# Autodesk Inventor assembly: boardstack
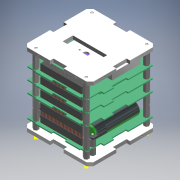
[picture p0: Inventor's stored thumbnail of the model, 180x180]
Saved by Autodesk Inventor 2022.3 (Build 263350000, 350)
## iProperties
Created: 2021-10-07
Part Number: boardstack
Document SubType Name: Assembly
Designer: Bowen O'Steen
Mass: 647.8 g
Surface Area: 2149.86 cm^2
Volume: 273.038 cm^3
Density: 2.37256 g/cm^3
Author: Bowen O'Steen
## Documents named in this file (11)
- C:\Users\gwhen\OneDrive\Documents\Vault\Engineering Data\MemeSat\Assembly\boardstack.iam
- C:\Users\gwhen\OneDrive\Desktop\Vault\Designs\MEMESat\MemeSat\Engineering Data\MemeSat\Subsystems\LFR\fullLFRboard.iam
- C:\Users\gwhen\OneDrive\Desktop\Vault\Designs\MEMESat\MemeSat\Engineering Data\MemeSat\Subsystems\OBC\OBC.iam
- C:\Users\gwhen\OneDrive\Desktop\Vault\Designs\MEMESat\MemeSat\Engineering Data\MemeSat\Subsystems\BoBa\BoBa.iam
- C:\Users\gwhen\OneDrive\Desktop\Vault\Designs\MEMESat\MemeSat\Engineering Data\MemeSat\Internal Components\pc104standoff.ipt
- C:\Users\gwhen\OneDrive\Desktop\Vault\Designs\MEMESat\MemeSat\Engineering Data\MemeSat\Subsystems\fullPCIconnector.iam
- C:\Users\gwhen\OneDrive\Desktop\Vault\Designs\MEMESat\MemeSat\Engineering Data\MemeSat\Subsystems\blankPC104plus.iam
- C:\Users\gwhen\OneDrive\Desktop\Vault\Designs\MEMESat\MemeSat\Engineering Data\MemeSat\Internal Components\stackframesupport.ipt
- C:\Users\gwhen\OneDrive\Desktop\Vault\Designs\MEMESat\MemeSat\Engineering Data\MemeSat\Internal Components\stackframesupportbottom.ipt
- C:\Users\gwhen\OneDrive\Desktop\Vault\Designs\MEMESat\MemeSat\Engineering Data\MemeSat\Internal Components\pc104standoffTEMP.ipt
- C:\Users\gwhen\OneDrive\Desktop\Vault\Designs\MEMESat\MemeSat\Engineering Data\MemeSat\Internal Components\pcBOBAstandoff.ipt
## Components (43 placed, 9 different names)
1. fullLFRboard:1 [sub-assembly] — Flush:1, Flush:2, Flush:3, Mate:1, Mate:2, Mate:3, Mate:4, Mate:5, Mate:6, Mate:7, Mate:8, Mate:46, Mate:47, Mate:61
2. OBC:1 [sub-assembly] — Mate:9, Mate:10, Mate:11, Mate:12, Mate:13, Mate:14, Mate:15, Mate:16, Mate:17, Mate:18, Mate:19, Angle:5, Angle:6, Angle:7, Angle:8
3. blankPC104plus:1 [sub-assembly] — Mate:20, Mate:21, Mate:22, Mate:23, Mate:24, Mate:25, Mate:26, Mate:31, Mate:32, Mate:33, Mate:34, Mate:43, Mate:44, Mate:45, Angle:9, Angle:10, Angle:11, Angle:12, Flush:6, Angle:13, Angle:20
4. pc104standoff:1 — Mate:1, Mate:8, Angle:5, Flush:8
5. pc104standoff:2 — Mate:2, Mate:7, Mate:9, Mate:10, Angle:6, Flush:9
6. pc104standoff:3 — Mate:3, Mate:5, Mate:11, Angle:8, Flush:10, Mate:60
7. pc104standoff:4 — Mate:4, Mate:6, Angle:7, Flush:7
8. pc104standoff:5 — Mate:12, Mate:17, Mate:20, Mate:22, Angle:10
9. pc104standoff:6 — Mate:13, Mate:16, Mate:21, Angle:9
10. pc104standoff:7 — Mate:14, Mate:19, Angle:11
11. pc104standoff:8 — Mate:15, Mate:18, Angle:12
12. pc104standoff:9 — Mate:26, Mate:30, Mate:32, Mate:37, Angle:13, Angle:14
13. pc104standoff:10 — Mate:24, Mate:28, Mate:34, Mate:36, Angle:23
14. pc104standoff:11 — Mate:23, Mate:29, Mate:31, Mate:35, Angle:20
15. pc104standoff:12 — Mate:25, Mate:27, Mate:33, Mate:38, Angle:24
16. pc104standoff:13 — Mate:27, Mate:38, Flush:14, Angle:24
17. pc104standoff:14 — Mate:28, Mate:36, Flush:11, Angle:23
18. pc104standoff:15 — Mate:29, Mate:35, Flush:12, Angle:21
19. pc104standoff:16 — Mate:30, Mate:37, Flush:13, Mate:50, Angle:14
20. fullPCIconnector:1 [sub-assembly] — Mate:43, Mate:44, Mate:45, Flush:5
21. stackframesupport:2 — Insert:1, Insert:2, Insert:3
22. stackframesupportbottom:1 — Insert:7, Insert:8, Insert:9, Insert:10, Insert:11, Mate:54, Mate:55
23. pc104standoff:21
24. pc104standoff:22
25. pc104standoff:23
26. pc104standoff:24
27. BoBa:1 [sub-assembly] — Flush:5, Flush:6, Insert:4, Insert:5, Insert:6, Mate:49, Mate:50, Mate:51, Angle:15, Angle:16, Mate:53, Angle:17, Mate:57, Mate:59, Angle:18, Angle:19, Angle:21, Angle:22
28. pcLFRstandoff:1 — Insert:1, Flush:7
29. pcLFRstandoff:2 — Insert:2, Flush:8, Mate:47
30. pcLFRstandoff:3 — Insert:3, Flush:9, Mate:46
31. pcLFRstandoff:4 — Flush:10, Mate:60, Mate:61
32. pcLFRstandoff:5 — Insert:4, Flush:11, Insert:7, Flush:15
33. pcLFRstandoff:6 — Insert:6, Flush:13
34. pcLFRstandoff:7 — Flush:14, Flush:16, Mate:54, Mate:55
35. pcLFRstandoff:8 — Insert:5, Flush:12, Angle:22
36. pcLFRstandoff:9 — Insert:8, Flush:15, Mate:56
37. pcLFRstandoff:10 — Insert:9, Flush:16, Mate:52
38. pcLFRstandoff:11 — Insert:11, Mate:58, Angle:19
39. pcLFRstandoff:12 — Insert:10, Mate:48, Mate:51, Angle:16
40. pcLFRstandoff:13 — Mate:48, Mate:49, Angle:15
41. pcLFRstandoff:14 — Mate:52, Mate:53, Angle:17
42. pcLFRstandoff:15 — Mate:56, Mate:57
43. pcLFRstandoff:16 — Mate:58, Mate:59, Angle:18
## Relationships (103: Mate 57, Angle 20, Flush 15, Insert 11)
- Flush:1: fullLFRboard:1
- Flush:2: fullLFRboard:1
- Flush:3: fullLFRboard:1
- Mate:1: fullLFRboard:1 ↔ pc104standoff:1
- Mate:2: fullLFRboard:1 ↔ pc104standoff:2
- Mate:3: fullLFRboard:1 ↔ pc104standoff:3
- Mate:4: fullLFRboard:1 ↔ pc104standoff:4
- Mate:5: fullLFRboard:1 ↔ pc104standoff:3
- Mate:6: fullLFRboard:1 ↔ pc104standoff:4
- Mate:7: fullLFRboard:1 ↔ pc104standoff:2
- Mate:8: fullLFRboard:1 ↔ pc104standoff:1
- Mate:9: OBC:1 ↔ pc104standoff:2
- Mate:10: OBC:1 ↔ pc104standoff:2
- Mate:11: OBC:1 ↔ pc104standoff:3
- Mate:12: OBC:1 ↔ pc104standoff:5
- Mate:13: OBC:1 ↔ pc104standoff:6
- Mate:14: OBC:1 ↔ pc104standoff:7
- Mate:15: OBC:1 ↔ pc104standoff:8
- Mate:16: OBC:1 ↔ pc104standoff:6
- Mate:17: OBC:1 ↔ pc104standoff:5
- Mate:18: OBC:1 ↔ pc104standoff:8
- Mate:19: OBC:1 ↔ pc104standoff:7
- Mate:20: blankPC104plus:1 ↔ pc104standoff:5
- Mate:21: blankPC104plus:1 ↔ pc104standoff:6
- Mate:22: blankPC104plus:1 ↔ pc104standoff:5
- Mate:23: blankPC104plus:1 ↔ pc104standoff:11
- Mate:24: blankPC104plus:1 ↔ pc104standoff:10
- Mate:25: blankPC104plus:1 ↔ pc104standoff:12
- Mate:26: blankPC104plus:1 ↔ pc104standoff:9
- Mate:27: pc104standoff:12 ↔ pc104standoff:13
- Mate:28: pc104standoff:10 ↔ pc104standoff:14
- Mate:29: pc104standoff:11 ↔ pc104standoff:15
- Mate:30: pc104standoff:9 ↔ pc104standoff:16
- Mate:31: blankPC104plus:1 ↔ pc104standoff:11
- Mate:32: blankPC104plus:1 ↔ pc104standoff:9
- Mate:33: blankPC104plus:1 ↔ pc104standoff:12
- Mate:34: blankPC104plus:1 ↔ pc104standoff:10
- Mate:35: pc104standoff:11 ↔ pc104standoff:15
- Mate:36: pc104standoff:10 ↔ pc104standoff:14
- Mate:37: pc104standoff:9 ↔ pc104standoff:16
- Mate:38: pc104standoff:12 ↔ pc104standoff:13
- Mate:43: blankPC104plus:1 ↔ fullPCIconnector:1
- Mate:44: blankPC104plus:1 ↔ fullPCIconnector:1
- Mate:45: blankPC104plus:1 ↔ fullPCIconnector:1
- Angle:5 (0 deg): OBC:1 ↔ pc104standoff:1
- Angle:6 (0 deg): OBC:1 ↔ pc104standoff:2
- Angle:7 (0 deg): OBC:1 ↔ pc104standoff:4
- Angle:8 (0 deg): OBC:1 ↔ pc104standoff:3
- Angle:9 (0 deg): blankPC104plus:1 ↔ pc104standoff:6
- Angle:10 (0 deg): blankPC104plus:1 ↔ pc104standoff:5
- Angle:11 (0 deg): blankPC104plus:1 ↔ pc104standoff:7
- Angle:12 (0 deg): blankPC104plus:1 ↔ pc104standoff:8
- Flush:5: fullPCIconnector:1 ↔ BoBa:1
- Flush:6: blankPC104plus:1 ↔ BoBa:1
- Insert:1: stackframesupport:2 ↔ pcLFRstandoff:1
- Flush:7: pc104standoff:4 ↔ pcLFRstandoff:1
- Insert:2: stackframesupport:2 ↔ pcLFRstandoff:2
- Flush:8: pc104standoff:1 ↔ pcLFRstandoff:2
- Insert:3: stackframesupport:2 ↔ pcLFRstandoff:3
- Flush:9: pc104standoff:2 ↔ pcLFRstandoff:3
- Flush:10: pc104standoff:3 ↔ pcLFRstandoff:4
- Mate:46: fullLFRboard:1 ↔ pcLFRstandoff:3
- Mate:47: fullLFRboard:1 ↔ pcLFRstandoff:2
- Insert:4: BoBa:1 ↔ pcLFRstandoff:5
- Flush:11: pc104standoff:14 ↔ pcLFRstandoff:5
- Insert:5: BoBa:1 ↔ pcLFRstandoff:8
- Flush:12: pc104standoff:15 ↔ pcLFRstandoff:8
- Insert:6: BoBa:1 ↔ pcLFRstandoff:6
- Flush:13: pc104standoff:16 ↔ pcLFRstandoff:6
- Flush:14: pc104standoff:13 ↔ pcLFRstandoff:7
- Insert:7: stackframesupportbottom:1 ↔ pcLFRstandoff:5
- Insert:8: stackframesupportbottom:1 ↔ pcLFRstandoff:9
- Flush:15: pcLFRstandoff:5 ↔ pcLFRstandoff:9
- Insert:9: stackframesupportbottom:1 ↔ pcLFRstandoff:10
- Flush:16: pcLFRstandoff:7 ↔ pcLFRstandoff:10
- Insert:10: stackframesupportbottom:1 ↔ pcLFRstandoff:12
- Insert:11: stackframesupportbottom:1 ↔ pcLFRstandoff:11
- Mate:48: pcLFRstandoff:12 ↔ pcLFRstandoff:13
- Mate:49: BoBa:1 ↔ pcLFRstandoff:13
- Mate:50: pc104standoff:16 ↔ BoBa:1
- Angle:13 (0 deg): blankPC104plus:1 ↔ pc104standoff:9
- Angle:14 (0 deg): pc104standoff:9 ↔ pc104standoff:16
- Mate:51: BoBa:1 ↔ pcLFRstandoff:12
- Angle:15 (0 deg): BoBa:1 ↔ pcLFRstandoff:13
- Angle:16 (0 deg): BoBa:1 ↔ pcLFRstandoff:12
- Mate:52: pcLFRstandoff:10 ↔ pcLFRstandoff:14
- Mate:53: BoBa:1 ↔ pcLFRstandoff:14
- Angle:17 (0 deg): BoBa:1 ↔ pcLFRstandoff:14
- Mate:54: stackframesupportbottom:1 ↔ pcLFRstandoff:7
- Mate:55: stackframesupportbottom:1 ↔ pcLFRstandoff:7
- Mate:56: pcLFRstandoff:9 ↔ pcLFRstandoff:15
- Mate:57: BoBa:1 ↔ pcLFRstandoff:15
- Mate:58: pcLFRstandoff:11 ↔ pcLFRstandoff:16
- Mate:59: BoBa:1 ↔ pcLFRstandoff:16
- Angle:18 (0 deg): BoBa:1 ↔ pcLFRstandoff:16
- Angle:19 (0 deg): BoBa:1 ↔ pcLFRstandoff:11
- Angle:20 (0 deg): blankPC104plus:1 ↔ pc104standoff:11
- Angle:21 (0 deg): pc104standoff:15 ↔ BoBa:1
- Angle:22 (0 deg): BoBa:1 ↔ pcLFRstandoff:8
- Angle:23 (0 deg): pc104standoff:10 ↔ pc104standoff:14
- Angle:24 (0 deg): pc104standoff:12 ↔ pc104standoff:13
- Mate:60: pc104standoff:3 ↔ pcLFRstandoff:4
- Mate:61: fullLFRboard:1 ↔ pcLFRstandoff:4
